# Autodesk Inventor assembly: IR
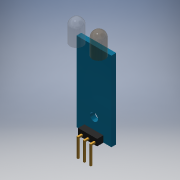
[picture p0: Inventor's stored thumbnail of the model, 180x180]
Saved by Autodesk Inventor 2018 (Build 220112000, 112)
## iProperties
Created: 2018-01-13
Part Number: IR
Document SubType Name: Assembly
Designer: Kyle-HP
Author: Kyle-HP
## Documents named in this file (6)
- C:\Users\Kyle-HP\Documents\Hackathon-2018\Inventor\Robot\IR.iam
- C:\Users\Kyle-HP\Documents\Hackathon-2018\Inventor\Robot\IRBoard.ipt
- C:\Users\Kyle-HP\Documents\Hackathon-2018\Inventor\Robot\IRIOBase.ipt
- C:\Users\Kyle-HP\Documents\Hackathon-2018\Inventor\Robot\IRIOPin.ipt
- C:\Users\Kyle-HP\Documents\Hackathon-2018\Inventor\Robot\IRRX.ipt
- C:\Users\Kyle-HP\Documents\Hackathon-2018\Inventor\Robot\IRTX.ipt
## Components (7 placed, 5 different names)
1. IRBoard:1 — Mate:1, Flush:1, Flush:2, Mate:5, Tangent:1, Tangent:2, Mate:6, Tangent:3, Tangent:4
2. IRIOBase:1 — Mate:1, Flush:1, Flush:2, Mate:2, Flush:3, Flush:4, Mate:3, Flush:5, Flush:6, Mate:4, Flush:7, Flush:8
3. IRIOPin:1 — Mate:2, Flush:3, Flush:4
4. IRIOPin:2 — Mate:3, Flush:5, Flush:6
5. IRIOPin:3 — Mate:4, Flush:7, Flush:8
6. IRRX:1 — Mate:5, Tangent:1, Tangent:2
7. IRTX:1 — Mate:6, Tangent:3, Tangent:4
## Relationships (18: Flush 8, Mate 6, Tangent 4)
- Mate:1: IRBoard:1 ↔ IRIOBase:1
- Flush:1: IRBoard:1 ↔ IRIOBase:1
- Flush:2 (3.175 mm): IRBoard:1 ↔ IRIOBase:1
- Mate:2: IRIOBase:1 ↔ IRIOPin:1
- Flush:3 (1.27 mm): IRIOBase:1 ↔ IRIOPin:1
- Flush:4 (1.27 mm): IRIOBase:1 ↔ IRIOPin:1
- Mate:3: IRIOBase:1 ↔ IRIOPin:2
- Flush:5 (3.81 mm): IRIOBase:1 ↔ IRIOPin:2
- Flush:6 (1.27 mm): IRIOBase:1 ↔ IRIOPin:2
- Mate:4: IRIOBase:1 ↔ IRIOPin:3
- Flush:7 (6.35 mm): IRIOBase:1 ↔ IRIOPin:3
- Flush:8 (1.27 mm): IRIOBase:1 ↔ IRIOPin:3
- Mate:5: IRBoard:1 ↔ IRRX:1
- Tangent:1: IRBoard:1 ↔ IRRX:1
- Tangent:2: IRBoard:1 ↔ IRRX:1
- Mate:6: IRBoard:1 ↔ IRTX:1
- Tangent:3: IRBoard:1 ↔ IRTX:1
- Tangent:4: IRBoard:1 ↔ IRTX:1
